# Autodesk Inventor assembly: Assembly4
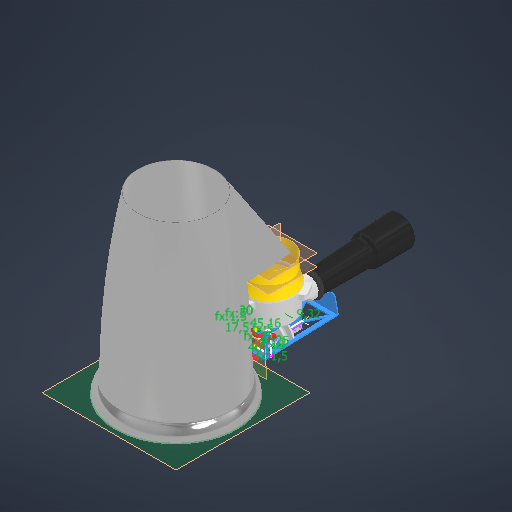
[picture p0: Inventor's stored thumbnail of the model, 512x512]
Saved by Autodesk Inventor 2026 (Build 300175000, 175)
## iProperties
Created: 2025-04-29
Part Number: Assembly4
Document SubType Name: Assembly
Designer: Paul Juschitz
Author: Paul Juschitz
## Documents named in this file (7)
- C:\Users\Paul Juschitz\Documents\private\m5_GBW_mod\M5_GBW_mod\CAD\Assembly4.iam
- C:\Users\Paul Juschitz\Documents\private\m5_GBW_mod\M5_GBW_mod\CAD\m2m_shell.ipt
- C:\Users\Paul Juschitz\Documents\private\m5_GBW_mod\M5_GBW_mod\CAD\load_cell.ipt
- C:\Users\Paul Juschitz\Documents\private\m5_GBW_mod\M5_GBW_mod\CAD\my_portafilter_holder_7.ipt
- C:\Users\Paul Juschitz\Documents\private\m5_GBW_mod\M5_GBW_mod\CAD\downloads\portafilter\BES870XL Portafilter\BES870XL Portafilter\BES870XL Portafilter_assembled.iam
- C:\Users\Paul Juschitz\Documents\private\m5_GBW_mod\M5_GBW_mod\CAD\mock_dosing_funnel.ipt
- C:\Users\Paul Juschitz\Documents\private\m5_GBW_mod\M5_GBW_mod\CAD\load_cell_bracket_2.ipt
## Components (6 placed, 6 different names)
1. m2m_shell:1 — Flush:1, Mate:8, Mate:11
2. load_cell:1 — Mate:5, Mate:6, Mate:9, Cylindrical:1, Cylindrical:2, Mate:10
3. my_portafilter_holder_7:1 — Mate:5, Mate:6, Tangent:2
4. BES870XL Portafilter_assembled:1 [sub-assembly] — Flush:1, Tangent:2, Mate:7
5. mock_dosing_funnel:1 — Mate:7
6. load_cell_bracket_2:1 — Mate:8, Mate:9, Cylindrical:1, Cylindrical:2, Mate:10, Mate:11
## Relationships (11: Mate 7, CylindricalJoint 2, Flush 1, Tangent 1)
- Mate:5: load_cell:1 ↔ my_portafilter_holder_7:1
- Mate:6: load_cell:1 ↔ my_portafilter_holder_7:1
- Flush:1: m2m_shell:1 ↔ BES870XL Portafilter_assembled:1
- Tangent:2: my_portafilter_holder_7:1 ↔ BES870XL Portafilter_assembled:1
- Mate:7: BES870XL Portafilter_assembled:1 ↔ mock_dosing_funnel:1
- Mate:8: m2m_shell:1 ↔ load_cell_bracket_2:1
- Mate:9: load_cell:1 ↔ load_cell_bracket_2:1
- Cylindrical:1: load_cell:1 ↔ load_cell_bracket_2:1
- Cylindrical:2: load_cell:1 ↔ load_cell_bracket_2:1
- Mate:10: load_cell:1 ↔ load_cell_bracket_2:1
- Mate:11: m2m_shell:1 ↔ load_cell_bracket_2:1
